# Autodesk Inventor assembly: Assembly1
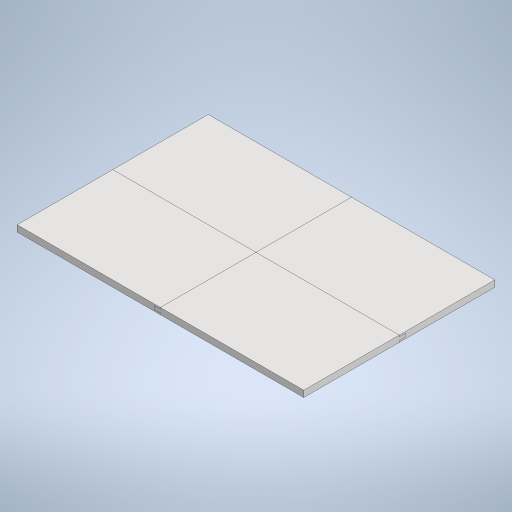
[picture p0: Inventor's stored thumbnail of the model, 512x512]
Saved by Autodesk Inventor 2024 (Build 280153000, 153)
## iProperties
Created: 2024-12-30
Part Number: Assembly1
Document SubType Name: Assembly
Designer: mtidd
Author: mtidd
## Documents named in this file (4)
- C:\Users\mtidd\OneDrive\Desktop\H2A\CAD\Trash Storage Unit\Assembly1.iam
- C:\Users\mtidd\OneDrive\Desktop\H2A\CAD\Trash Storage Unit\TSU_Baseplate_Female.ipt
- C:\Users\mtidd\OneDrive\Desktop\H2A\CAD\Trash Storage Unit\TSU_Baseplate_Male.ipt
- C:\Users\mtidd\OneDrive\Desktop\H2A\CAD\Trash Storage Unit\TSU_Baseplate_Male_Cut.ipt
## Components (4 placed, 3 different names)
1. TSU_Baseplate_Female:1 — Mate:1, Mate:2
2. TSU_Baseplate_Male:1 — Mate:1, Mate:2, Mate:3, Mate:4
3. TSU_Baseplate_Female:2 — Mate:3, Mate:4, Mate:5, Mate:6
4. TSU_Baseplate_Male_Cut:1 — Mate:5, Mate:6
## Relationships (6: Mate 6)
- Mate:1: TSU_Baseplate_Female:1 ↔ TSU_Baseplate_Male:1
- Mate:2: TSU_Baseplate_Female:1 ↔ TSU_Baseplate_Male:1
- Mate:3: TSU_Baseplate_Male:1 ↔ TSU_Baseplate_Female:2
- Mate:4: TSU_Baseplate_Male:1 ↔ TSU_Baseplate_Female:2
- Mate:5: TSU_Baseplate_Female:2 ↔ TSU_Baseplate_Male_Cut:1
- Mate:6: TSU_Baseplate_Female:2 ↔ TSU_Baseplate_Male_Cut:1
